# Autodesk Inventor assembly: Shoulder
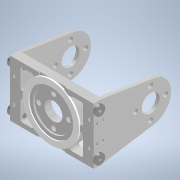
[picture p0: Inventor's stored thumbnail of the model, 180x180]
Saved by Autodesk Inventor 2020.4 (Build 244396000, 396)
## iProperties
Created: 2021-09-24
Part Number: Shoulder
Document SubType Name: Assembly
Designer: Masato Kubotera
Mass: 26.1068 g
Surface Area: 95.2903 cm^2
Volume: 8.79774 cm^3
Density: 2.96744 g/cm^3
Author: Masato Kubotera
## Documents named in this file (5)
- C:\Users\Masato\Documents\Inventor\CIT Brains_Inventor\OpenPlatform_ver3_0\UpperBody\Arm\Shoulder.iam
- C:\Users\Masato\Documents\Inventor\CIT Brains_Inventor\OpenPlatform_ver3_0\UpperBody\Arm\Shoulder_vertical_frame_01.ipt
- C:\Users\Masato\Documents\Inventor\CIT Brains_Inventor\OpenPlatform_ver3_0\UpperBody\Arm\Shoulder_vertical_frame_02.ipt
- C:\Users\Masato\Documents\Inventor\CIT Brains_Inventor\OpenPlatform_ver3_0\Ready_Made\Screw\M3-6.ipt
- C:\Users\Masato\Documents\Inventor\CIT Brains_Inventor\OpenPlatform_ver3_0\Ready_Made\TT-2532-10.ipt
## Components (8 placed, 4 different names)
1. Shoulder_vertical_frame_01:1 — 挿入:1, 挿入:2, 挿入:3, 挿入:4, 挿入:9
2. Shoulder_vertical_frame_02:1 — 挿入:1, 挿入:2, 挿入:7, 挿入:8
3. Shoulder_vertical_frame_02:2 — 挿入:3, 挿入:4, 挿入:5, 挿入:6
4. M3-6:1 — 挿入:5
5. M3-6:2 — 挿入:6
6. M3-6:3 — 挿入:7
7. M3-6:4 — 挿入:8
8. TT-2532-10:1 — 挿入:9
## Relationships (9: Insert 9)
- 挿入:1 [Insert]: Shoulder_vertical_frame_01:1 ↔ Shoulder_vertical_frame_02:1
- 挿入:2 [Insert]: Shoulder_vertical_frame_01:1 ↔ Shoulder_vertical_frame_02:1
- 挿入:3 [Insert]: Shoulder_vertical_frame_01:1 ↔ Shoulder_vertical_frame_02:2
- 挿入:4 [Insert]: Shoulder_vertical_frame_01:1 ↔ Shoulder_vertical_frame_02:2
- 挿入:5 [Insert]: Shoulder_vertical_frame_02:2 ↔ M3-6:1
- 挿入:6 [Insert]: Shoulder_vertical_frame_02:2 ↔ M3-6:2
- 挿入:7 [Insert]: Shoulder_vertical_frame_02:1 ↔ M3-6:3
- 挿入:8 [Insert]: Shoulder_vertical_frame_02:1 ↔ M3-6:4
- 挿入:9 [Insert]: Shoulder_vertical_frame_01:1 ↔ TT-2532-10:1
